# Autodesk Inventor assembly: LED Filament Assembly
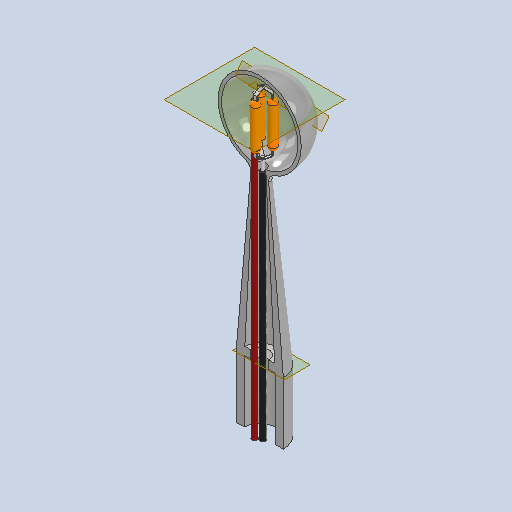
[picture p0: Inventor's stored thumbnail of the model, 512x512]
Saved by Autodesk Inventor 2022 (Build 260153000, 153)
## iProperties
Created: 2022-02-02
Part Number: LED Filament Assembly
Document SubType Name: Assembly
Designer: tecware
Author: tecware
## Documents named in this file (5)
- C:\Users\tecware\Documents\git\calibrationKit\LED Filament Assembly\LED Filament Assembly.iam
- C:\Users\tecware\Documents\git\calibrationKit\components_shared\LED Single Filament.ipt
- C:\Users\tecware\Documents\git\calibrationKit\components_shared\wire-red.ipt
- C:\Users\tecware\Documents\git\calibrationKit\components_shared\wire-black.ipt
- C:\Users\tecware\Documents\git\calibrationKit\T-wand\markerWithRodEnd.ipt
## Components (6 placed, 4 different names)
1. LED Single Filament:1 — Mate:1
2. LED Single Filament:2
3. LED Single Filament:3
4. wire-red:1 — Mate:1
5. wire-black:1
6. markerWithRodEnd:1
## Relationships (1: Mate 1)
- Mate:1: LED Single Filament:1 ↔ wire-red:1
